# Autodesk Inventor assembly: Assembly4
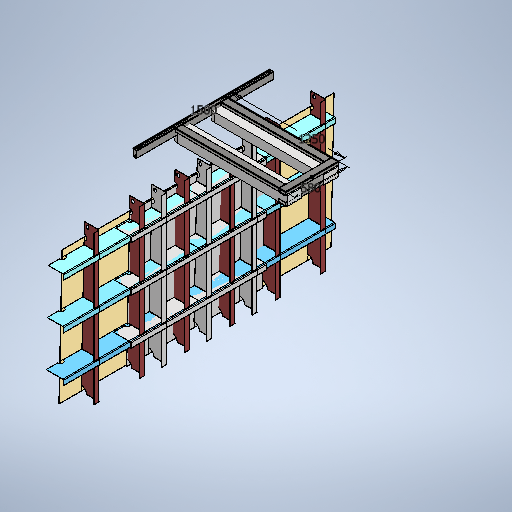
[picture p0: Inventor's stored thumbnail of the model, 512x512]
Saved by Autodesk Inventor 2026.2 (Build 302298010, 298A)
## iProperties
Created: 2026-06-02
Part Number: Assembly4
Document SubType Name: Assembly
Designer: admin
Author: admin
## Documents named in this file (5)
- C:\Users\admin\Documents\Inventor\GBK-Gubkinskiy\Assembly4.iam
- C:\Users\admin\Documents\Inventor\GBK-Gubkinskiy\ASY GBK 1120 long wall shield 2.iam
- C:\Users\admin\Documents\Inventor\GBK-Gubkinskiy\ASY GBK 1110 long wall shield 1.iam
- C:\Users\admin\Documents\Inventor\GBK-Gubkinskiy\pallet jack dummy.ipt
- C:\Users\admin\Documents\Inventor\GBK-Gubkinskiy\Траверса.iam
## Components (4 placed, 4 different names)
1. 02 ASY GBK wall shield 1.1.2:1 [sub-assembly] — Flush:4
2. ASY GBK 1110 long wall shield 1:1 [sub-assembly] — Flush:3
3. pallet jack dummy:1 — Mate:1, Flush:1, Flush:2, Flush:6, Mate:2
4. Траверса:1 [sub-assembly] — Flush:6, Mate:2
## Relationships (7: Flush 5, Mate 2)
- Mate:1 (2000 mm): pallet jack dummy:1
- Flush:1: pallet jack dummy:1
- Flush:2: pallet jack dummy:1
- Flush:3: ASY GBK 1110 long wall shield 1:1
- Flush:4: 02 ASY GBK wall shield 1.1.2:1
- Flush:6: pallet jack dummy:1 ↔ Траверса:1
- Mate:2: pallet jack dummy:1 ↔ Траверса:1
